# Autodesk Inventor assembly: Compute Node Assembly
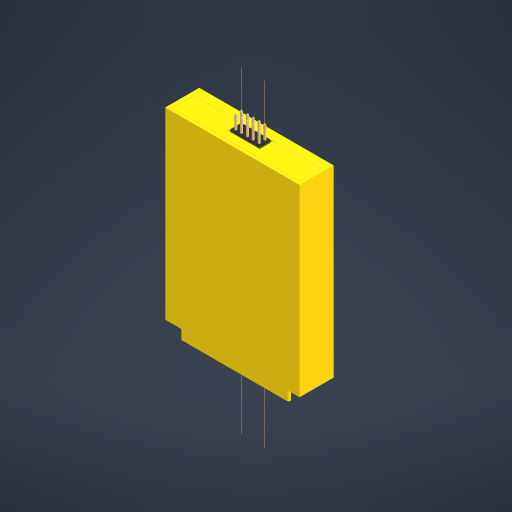
[picture p0: Inventor's stored thumbnail of the model, 512x512]
Saved by Autodesk Inventor 2024 (Build 280153000, 153)
## iProperties
Created: 2025-04-21
Part Number: Compute Node Assembly
Document SubType Name: Assembly
Designer: apodd
Author: apodd
## Documents named in this file (4)
- C:\Users\apodd\Desktop\BoilerNet CAD Files\Assemblies\Compute Node Assembly.iam
- C:\Users\apodd\Desktop\BoilerNet CAD Files\Parts\Compute Node Enclosure.ipt
- C:\Users\apodd\Desktop\BoilerNet CAD Files\Parts\Compute Node.ipt
- C:\Users\apodd\Desktop\BoilerNet CAD Files\Parts\Compute Node Lid.ipt
## Components (3 placed, 3 different names)
1. Compute Node Enclosure:1 — Mate:1, Mate:2, Mate:3, Flush:1, Flush:2
2. Compute Node:1 — Mate:1, Mate:2, Mate:3, Flush:3
3. Compute Node Lid:1 — Flush:1, Flush:2
## Relationships (6: Mate 3, Flush 3)
- Mate:1: Compute Node Enclosure:1 ↔ Compute Node:1
- Mate:2: Compute Node Enclosure:1 ↔ Compute Node:1
- Mate:3 (0.3514 mm): Compute Node Enclosure:1 ↔ Compute Node:1
- Flush:1: Compute Node Enclosure:1 ↔ Compute Node Lid:1
- Flush:2: Compute Node Enclosure:1 ↔ Compute Node Lid:1
- Flush:3 (-0.4 mm): Compute Node:1
